# Autodesk Inventor assembly: Cryostat
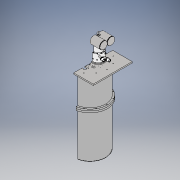
[picture p0: Inventor's stored thumbnail of the model, 180x180]
Saved by Autodesk Inventor 2018 (Build 220112000, 112)
## iProperties
Created: 2018-10-10
Part Number: Cryostat
Document SubType Name: Assembly
Designer: Admin
Author: Admin
## Documents named in this file (9)
- C:\Users\freyja\Documents\Cryorefrigerator\CAD\Cryostat.iam
- C:\Users\freyja\Documents\Cryorefrigerator\CAD\External Models\CH40415 24JUL14 C.ipt
- C:\Users\freyja\Documents\Cryorefrigerator\CAD\vacuum jacket long.ipt
- C:\Users\freyja\Documents\Cryorefrigerator\CAD\vacuum jacket.ipt
- C:\Users\freyja\Documents\Cryorefrigerator\CAD\Top Plate V2.2.ipt
- C:\Users\freyja\Documents\Cryorefrigerator\CAD\55K stage.ipt
- C:\Users\freyja\Documents\Cryorefrigerator\CAD\sheild stop.ipt
- C:\Users\freyja\Documents\Cryorefrigerator\CAD\55K shield sheet.ipt
- C:\Users\freyja\Documents\Cryorefrigerator\CAD\2K8 stage.ipt
## Components (8 placed, 8 different names)
1. Top Plate V2.2:1 — Mate:16, Mate:18, Mate:19, Mate:20, Mate:21, Mate:26
2. CH40415 24JUL14 C:1 — Mate:16, Mate:18, Mate:26, Mate:27, Mate:28, Mate:29, Mate:34, Mate:35, Mate:36
3. vacuum jacket long:1 — Mate:7, Mate:8, Mate:9
4. vacuum jacket:1 — Mate:7, Mate:8, Mate:9, Mate:19, Mate:20, Mate:21
5. 55K stage:1 — Mate:27, Mate:28, Mate:29, Mate:30, Mate:31, Mate:32
6. sheild stop:1 — Mate:30, Mate:31, Mate:33
7. 55K shield sheet:1 — Mate:32, Mate:33
8. 2K8 stage:1 — Mate:34, Mate:35, Mate:36
## Relationships (19: Mate 19)
- Mate:7: vacuum jacket long:1 ↔ vacuum jacket:1
- Mate:8: vacuum jacket long:1 ↔ vacuum jacket:1
- Mate:9: vacuum jacket long:1 ↔ vacuum jacket:1
- Mate:16: Top Plate V2.2:1 ↔ CH40415 24JUL14 C:1
- Mate:18: Top Plate V2.2:1 ↔ CH40415 24JUL14 C:1
- Mate:19: Top Plate V2.2:1 ↔ vacuum jacket:1
- Mate:20: Top Plate V2.2:1 ↔ vacuum jacket:1
- Mate:21: Top Plate V2.2:1 ↔ vacuum jacket:1
- Mate:26: Top Plate V2.2:1 ↔ CH40415 24JUL14 C:1
- Mate:27: CH40415 24JUL14 C:1 ↔ 55K stage:1
- Mate:28: CH40415 24JUL14 C:1 ↔ 55K stage:1
- Mate:29: CH40415 24JUL14 C:1 ↔ 55K stage:1
- Mate:30: 55K stage:1 ↔ sheild stop:1
- Mate:31: 55K stage:1 ↔ sheild stop:1
- Mate:32: 55K stage:1 ↔ 55K shield sheet:1
- Mate:33: sheild stop:1 ↔ 55K shield sheet:1
- Mate:34: CH40415 24JUL14 C:1 ↔ 2K8 stage:1
- Mate:35: CH40415 24JUL14 C:1 ↔ 2K8 stage:1
- Mate:36: CH40415 24JUL14 C:1 ↔ 2K8 stage:1
